# Autodesk Inventor assembly: KexT16TX
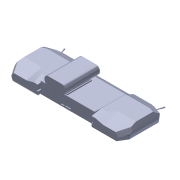
[picture p0: Inventor's stored thumbnail of the model, 180x180]
Saved by Autodesk Inventor 2019.4 (Build 234330000, 330)
## iProperties
Created: 2020-02-01
Part Number: KexT16TX
Document SubType Name: Assembly
Designer: xenial
Author: xenial
Sending System: SolidWorks 2016
Last Author: xenial
Last Saved: 2021-02-27
## Documents named in this file (4)
- C:\Users\xenial\Desktop\Kext16TX\KexT16TX.iam
- C:\Users\xenial\Desktop\Kext16TX\KexT16Main.iam
- C:\Users\xenial\Desktop\Kext16TX\HandleL.iam
- C:\Users\xenial\Desktop\Kext16TX\HandleR2.iam
## Components (3 placed, 3 different names)
1. KexT16Main:1 [sub-assembly] — Mate:1, Mate:2, Mate:3, Mate:4, Mate:5, Mate:6
2. HandleL:1 [sub-assembly] — Mate:4, Mate:5, Mate:6
3. HandleR2:1 [sub-assembly] — Mate:1, Mate:2, Mate:3
## Relationships (6: Mate 6)
- Mate:1: KexT16Main:1 ↔ HandleR2:1
- Mate:2: KexT16Main:1 ↔ HandleR2:1
- Mate:3: KexT16Main:1 ↔ HandleR2:1
- Mate:4: KexT16Main:1 ↔ HandleL:1
- Mate:5: KexT16Main:1 ↔ HandleL:1
- Mate:6: KexT16Main:1 ↔ HandleL:1
